# Autodesk Inventor assembly: A135
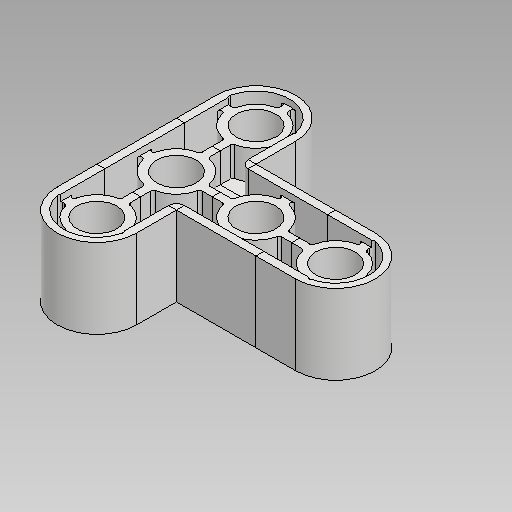
[picture p0: Inventor's stored thumbnail of the model, 512x512]
Saved by Autodesk Inventor 2020 (Build 240168000, 168)
## iProperties
Created: 2019-05-05
Part Number: A135
Document SubType Name: Assembly
Designer: Varga Daniel
Author: Varga Daniel
## Documents named in this file (4)
- C:\!_Dani\!_cloud\OneDrive\!_munka\Revolution\StructuralParts\Beams\Angled Beams\A90T.iam
- C:\!_Dani\!_cloud\OneDrive\!_munka\Revolution\StructuralParts\Beams\beam_single_end_part.ipt
- C:\!_Dani\!_cloud\OneDrive\!_munka\Revolution\StructuralParts\Beams\beam_single_inner_part.ipt
- C:\!_Dani\!_cloud\OneDrive\!_munka\Revolution\StructuralParts\Beams\Beam_T_base.ipt
## Components (5 placed, 3 different names)
1. Beam_T_base:1 — Mate:4, Flush:7, Flush:8, Flush:9, Flush:10, Flush:11, Flush:12, Mate:5, Mate:6
2. beam_single_end_part:1 — Flush:11, Flush:12, Mate:5
3. beam_single_end_part:2
4. beam_single_inner_part:4 — Mate:4, Flush:7, Flush:8
5. beam_single_end_part:3 — Flush:9, Flush:10, Mate:6
## Relationships (12: Flush 8, Mate 4)
- [Flush]: beam_single_end_part:2 ↔ beam_single_inner_part:4
- [Flush]: beam_single_end_part:2 ↔ beam_single_inner_part:4
- [Mate]: beam_single_end_part:2 ↔ beam_single_inner_part:4
- Mate:4: Beam_T_base:1 ↔ beam_single_inner_part:4
- Flush:7: Beam_T_base:1 ↔ beam_single_inner_part:4
- Flush:8: Beam_T_base:1 ↔ beam_single_inner_part:4
- Flush:9: Beam_T_base:1 ↔ beam_single_end_part:3
- Flush:10: Beam_T_base:1 ↔ beam_single_end_part:3
- Flush:11: Beam_T_base:1 ↔ beam_single_end_part:1
- Flush:12: Beam_T_base:1 ↔ beam_single_end_part:1
- Mate:5: Beam_T_base:1 ↔ beam_single_end_part:1
- Mate:6: Beam_T_base:1 ↔ beam_single_end_part:3
## Named parameters: d9_d0 = 0 mm, d10_d1 = 0 mm, d11_d2 = 0 mm
